# Autodesk Inventor assembly: Base
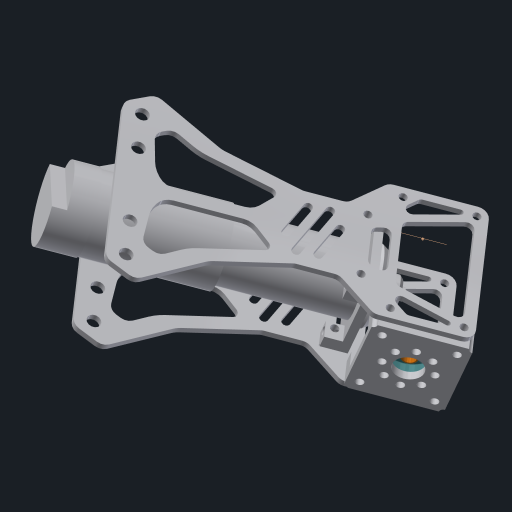
[picture p0: Inventor's stored thumbnail of the model, 512x512]
Saved by Autodesk Inventor 2023 (Build 270158000, 158)
## iProperties
Created: 2020-03-24
Part Number: Base
Document SubType Name: Assembly
Designer: valer
Mass: 4853.13 g
Surface Area: 3141.52 cm^2
Volume: 1403.99 cm^3
Density: 3.45667 g/cm^3
Author: valer
## Documents named in this file (11)
- C:\Users\valer\Desktop\str1ker\cad\ArmBase.iam
- C:\Users\valer\Desktop\str1ker\cad\external\ShoulderActuator\ShoulderActuator.ipt
- C:\Users\valer\Desktop\str1ker\cad\external\ShoulderMiterGear.ipt
- C:\Users\valer\Desktop\str1ker\cad\external\ShoulderActuator\ShoulderActuatorShaft.ipt
- C:\Users\valer\Desktop\str1ker\cad\external\ShoulderMotorMount.ipt
- C:\Users\valer\Desktop\str1ker\cad\external\PatternSpacer.ipt
- C:\Users\valer\Desktop\str1ker\cad\ShoulderBracket.ipt
- C:\Users\valer\Desktop\str1ker\cad\external\Potentiometer\Potentiometer.iam
- C:\Users\valer\Desktop\str1ker\cad\BaseBoundingBox.ipt
- C:\Users\valer\Desktop\str1ker\cad\PotentiometerCover.ipt
- C:\Users\valer\Documents\Inventor\Content Center Files\R2023\en-US\AS 1420\AS 1420 - 1973 - M3 x 6.ipt
## Components (21 placed, 10 different names)
1. ShoulderServo:1 — Mate:301, Mate:367, Mate:368
2. ShoulderMiterGear:1 — Mate:303, Mate:369
3. ShoulderServoShaft:1 — Mate:301, Mate:303, Mate:316, Mate:367
4. ShoulderMotorMount:1 — Mate:316, Mate:326, Mate:365, Mate:366, Mate:368, Mate:369
5. ShoulderMotorMount:2 — Mate:321, Mate:323, Mate:324, Mate:325, Mate:328, Mate:364, Mate:370, Mate:371
6. PatternSpacer:1 — Mate:321, Mate:363, Mate:370, Mate:371, Flush:1, Mate:375
7. ShoulderBracket:1 — Mate:323, Mate:324, Mate:325, Mate:365, Mate:366, Mate:373, Angle:3
8. ShoulderBracket:2 — Mate:326, Mate:328, Mate:359, Mate:360, Mate:361, Mate:364, Angle:4
9. ShoulderMotorMount:3 — Mate:359, Mate:360, Mate:361, Mate:372, Mate:373, Mate:374, Angle:2
10. Potentiometer:1 [sub-assembly] — Mate:372, Mate:374, Angle:2, Flush:3, Mate:376, Mate:377
11. BaseBoundingBox:1 — Flush:2, Mate:375, Angle:4
12. PotentiometerCover:1 — Flush:3
13. PotentiometerCover:2 — Mate:376, Mate:377, Insert:1, Insert:2, Insert:3, Insert:4, Insert:5, Insert:6, Insert:7, Insert:8
14. AS 1420 - Metric M3 x 6:1 — Insert:1
15. AS 1420 - Metric M3 x 6:2 — Insert:2
16. AS 1420 - Metric M3 x 6:3 — Insert:3
17. AS 1420 - Metric M3 x 6:4 — Insert:4
18. AS 1420 - Metric M3 x 6:5 — Insert:5
19. AS 1420 - Metric M3 x 6:6 — Insert:6
20. AS 1420 - Metric M3 x 6:7 — Insert:7
21. AS 1420 - Metric M3 x 6:8 — Insert:8
## Relationships (41: Mate 27, Insert 8, Flush 3, Angle 3)
- Mate:301: ShoulderServo:1 ↔ ShoulderServoShaft:1
- Mate:303: ShoulderMiterGear:1 ↔ ShoulderServoShaft:1
- Mate:316: ShoulderServoShaft:1 ↔ ShoulderMotorMount:1
- Mate:321: ShoulderMotorMount:2 ↔ PatternSpacer:1
- Mate:323: ShoulderMotorMount:2 ↔ ShoulderBracket:1
- Mate:324: ShoulderMotorMount:2 ↔ ShoulderBracket:1
- Mate:325: ShoulderMotorMount:2 ↔ ShoulderBracket:1
- Mate:326: ShoulderMotorMount:1 ↔ ShoulderBracket:2
- Mate:328: ShoulderMotorMount:2 ↔ ShoulderBracket:2
- Mate:359: ShoulderBracket:2 ↔ ShoulderMotorMount:3
- Mate:360: ShoulderBracket:2 ↔ ShoulderMotorMount:3
- Mate:361: ShoulderBracket:2 ↔ ShoulderMotorMount:3
- Mate:363: PatternSpacer:1
- Mate:364: ShoulderMotorMount:2 ↔ ShoulderBracket:2
- Mate:365: ShoulderMotorMount:1 ↔ ShoulderBracket:1
- Mate:366: ShoulderMotorMount:1 ↔ ShoulderBracket:1
- Mate:367 (-4 mm): ShoulderServo:1 ↔ ShoulderServoShaft:1
- Mate:368: ShoulderServo:1 ↔ ShoulderMotorMount:1
- Mate:369 (1 mm): ShoulderMiterGear:1 ↔ ShoulderMotorMount:1
- Mate:370: ShoulderMotorMount:2 ↔ PatternSpacer:1
- Mate:371: ShoulderMotorMount:2 ↔ PatternSpacer:1
- Mate:372: ShoulderMotorMount:3 ↔ Potentiometer:1
- Mate:373: ShoulderBracket:1 ↔ ShoulderMotorMount:3
- Flush:1: PatternSpacer:1
- Mate:374: ShoulderMotorMount:3 ↔ Potentiometer:1
- Angle:2 (0 deg): ShoulderMotorMount:3 ↔ Potentiometer:1
- Flush:2: BaseBoundingBox:1
- Angle:3 (0 deg): ShoulderBracket:1
- Mate:375: PatternSpacer:1 ↔ BaseBoundingBox:1
- Angle:4 (0 deg): ShoulderBracket:2 ↔ BaseBoundingBox:1
- Flush:3: Potentiometer:1 ↔ PotentiometerCover:1
- Mate:376: Potentiometer:1 ↔ PotentiometerCover:2
- Mate:377: Potentiometer:1 ↔ PotentiometerCover:2
- Insert:1: PotentiometerCover:2 ↔ AS 1420 - Metric M3 x 6:1
- Insert:2: PotentiometerCover:2 ↔ AS 1420 - Metric M3 x 6:2
- Insert:3: PotentiometerCover:2 ↔ AS 1420 - Metric M3 x 6:3
- Insert:4: PotentiometerCover:2 ↔ AS 1420 - Metric M3 x 6:4
- Insert:5: PotentiometerCover:2 ↔ AS 1420 - Metric M3 x 6:5
- Insert:6: PotentiometerCover:2 ↔ AS 1420 - Metric M3 x 6:6
- Insert:7: PotentiometerCover:2 ↔ AS 1420 - Metric M3 x 6:7
- Insert:8: PotentiometerCover:2 ↔ AS 1420 - Metric M3 x 6:8
